# Autodesk Inventor assembly: cas
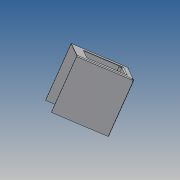
[picture p0: Inventor's stored thumbnail of the model, 180x180]
Saved by Autodesk Inventor 2017 (Build 210142000, 142)
## iProperties
Created: 2017-07-26
Part Number: cas
Document SubType Name: Assembly
Designer: leo
Author: leo
## Documents named in this file (2)
- C:\Users\Leo\Dropbox\multiactuador\cas.iam
- C:\Users\Leo\Dropbox\multiactuador\case\top.ipt
## Components (1 placed, 1 different names)
1. top:1 — Angle:1, Angle:2, Mate:1, Mate:2
## Relationships (4: Angle 2, Mate 2)
- Angle:1 (54.74 deg): top:1
- Angle:2 (54.74 deg): top:1
- Mate:1: top:1
- Mate:2: top:1
